# Autodesk Inventor assembly: 全底盘组
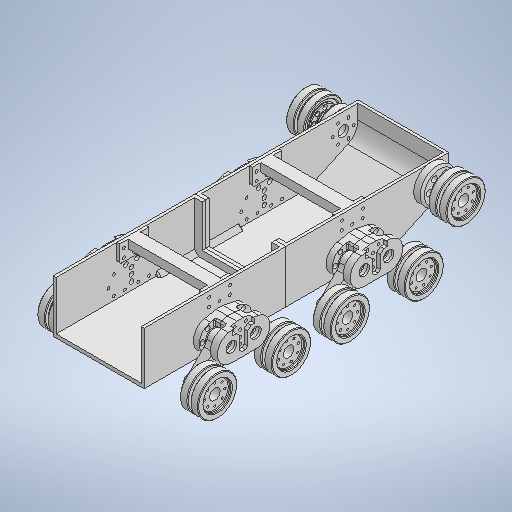
[picture p0: Inventor's stored thumbnail of the model, 512x512]
Saved by Autodesk Inventor 2025.1 (Build 291241000, 241)
## iProperties
Created: 2025-08-27
Part Number: 全底盘组
Document SubType Name: Assembly
Designer: Piw
Author: Piw
## Documents named in this file (3)
- C:\Users\22982\Desktop\急急急\Classis\全底盘组.iam
- C:\Users\22982\Desktop\急急急\Classis\后底盘组.iam
- C:\Users\22982\Desktop\急急急\Classis\前底盘组.iam
## Components (2 placed, 2 different names)
1. 后底盘组:1 [sub-assembly] — 配合:1, 表面齐平:1, 表面齐平:2
2. 前底盘组:1 [sub-assembly] — 配合:1, 表面齐平:1, 表面齐平:2
## Relationships (3: Flush 2, Mate 1)
- 配合:1 [Mate]: 后底盘组:1 ↔ 前底盘组:1
- 表面齐平:1 [Flush]: 后底盘组:1 ↔ 前底盘组:1
- 表面齐平:2 [Flush]: 后底盘组:1 ↔ 前底盘组:1
